# Autodesk Inventor assembly: Single_Burner_Stand_Assembly
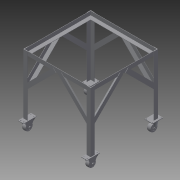
[picture p0: Inventor's stored thumbnail of the model, 180x180]
Saved by Autodesk Inventor 2014 (Build 180170000, 170)
## iProperties
Created: 2016-08-26
Part Number: Single_Burner_Stand_Assembly
Document SubType Name: Assembly
Designer: jmw3
Author: jmw3
## Documents named in this file (6)
- F:\NIST\Project_Files\FFT_Projects\UL_Drawings\Gas_Burner\Inventor_Parts\Single_Burner_Stand_Assembly.iam
- F:\NIST\Project_Files\FFT_Projects\UL_Drawings\Gas_Burner\Inventor_Parts\Single_Burner_Stand.ipt
- F:\NIST\Project_Files\FFT_Projects\UL_Drawings\Gas_Burner\Inventor_Parts\Rigid_Caster_Plate.ipt
- F:\NIST\Project_Files\FFT_Projects\UL_Drawings\Gas_Burner\Inventor_Parts\Swivel_Caster_Plate.ipt
- F:\NIST\Project_Files\FFT_Projects\UL_Drawings\Gas_Burner\Inventor_Parts\Rigid_Caster.ipt
- F:\NIST\Project_Files\FFT_Projects\UL_Drawings\Gas_Burner\Inventor_Parts\Swivel_Caster.ipt
## Components (9 placed, 5 different names)
1. Single_Burner_Stand:1 — Mate:1, Flush:1, Flush:2, Mate:2, Flush:4, Mate:3, Flush:5, Flush:6, Mate:4, Flush:8
2. Rigid_Caster_Plate:1 — Mate:2, Flush:3, Flush:4, Mate:5, Flush:9, Flush:10
3. Rigid_Caster_Plate:2 — Mate:1, Flush:1, Flush:2, Flush:3, Mate:6, Flush:11, Flush:12
4. Swivel_Caster_Plate:1 — Mate:3, Flush:5, Flush:6, Flush:7, Mate:7, Flush:13, Flush:14
5. Swivel_Caster_Plate:2 — Mate:4, Flush:7, Flush:8, Mate:8, Flush:15, Flush:16
6. Rigid_Caster:1 — Mate:5, Flush:9, Flush:10
7. Swivel_Caster:1 — Mate:7, Flush:13, Flush:14
8. Rigid_Caster:2 — Mate:6, Flush:11, Flush:12
9. Swivel_Caster:2 — Mate:8, Flush:15, Flush:16
## Relationships (24: Flush 16, Mate 8)
- Mate:1: Single_Burner_Stand:1 ↔ Rigid_Caster_Plate:2
- Flush:1 (-7.9375 mm): Single_Burner_Stand:1 ↔ Rigid_Caster_Plate:2
- Flush:2 (44.45 mm): Single_Burner_Stand:1 ↔ Rigid_Caster_Plate:2
- Mate:2: Single_Burner_Stand:1 ↔ Rigid_Caster_Plate:1
- Flush:3: Rigid_Caster_Plate:1 ↔ Rigid_Caster_Plate:2
- Flush:4 (-7.9375 mm): Single_Burner_Stand:1 ↔ Rigid_Caster_Plate:1
- Mate:3: Single_Burner_Stand:1 ↔ Swivel_Caster_Plate:1
- Flush:5 (-19.05 mm): Single_Burner_Stand:1 ↔ Swivel_Caster_Plate:1
- Flush:6 (-31.75 mm): Single_Burner_Stand:1 ↔ Swivel_Caster_Plate:1
- Mate:4: Single_Burner_Stand:1 ↔ Swivel_Caster_Plate:2
- Flush:7: Swivel_Caster_Plate:1 ↔ Swivel_Caster_Plate:2
- Flush:8 (-19.05 mm): Single_Burner_Stand:1 ↔ Swivel_Caster_Plate:2
- Mate:5: Rigid_Caster_Plate:1 ↔ Rigid_Caster:1
- Flush:9: Rigid_Caster_Plate:1 ↔ Rigid_Caster:1
- Flush:10: Rigid_Caster_Plate:1 ↔ Rigid_Caster:1
- Mate:6: Rigid_Caster_Plate:2 ↔ Rigid_Caster:2
- Flush:11: Rigid_Caster_Plate:2 ↔ Rigid_Caster:2
- Flush:12: Rigid_Caster_Plate:2 ↔ Rigid_Caster:2
- Mate:7: Swivel_Caster_Plate:1 ↔ Swivel_Caster:1
- Flush:13: Swivel_Caster_Plate:1 ↔ Swivel_Caster:1
- Flush:14: Swivel_Caster_Plate:1 ↔ Swivel_Caster:1
- Mate:8: Swivel_Caster_Plate:2 ↔ Swivel_Caster:2
- Flush:15: Swivel_Caster_Plate:2 ↔ Swivel_Caster:2
- Flush:16: Swivel_Caster_Plate:2 ↔ Swivel_Caster:2
